# Autodesk Inventor assembly: Assembly_Cube_Z-Focus_Objective_v3
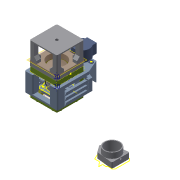
[picture p0: Inventor's stored thumbnail of the model, 180x180]
Saved by Autodesk Inventor 2019.4 (Build 234330000, 330)
## iProperties
Created: 2021-01-12
Part Number: Assembly_Cube_Z-Focus_Objective_v3
Document SubType Name: Assembly
Designer: diederichbenedict
Author: diederichbenedict
## Documents named in this file (5)
- C:\Users\diederichbenedict\Dropbox\Dokumente\Promotion\PROJECTS\UC2\02_CAD\INVENTOR\uc2_v3\Assembly_Cube_Z-Focus_Objective_v3.iam
- C:\Users\diederichbenedict\Dropbox\Dokumente\Promotion\PROJECTS\UC2\02_CAD\INVENTOR\uc2_v3\00_Olympus_40_1.3oil.ipt
- C:\Users\diederichbenedict\Dropbox\Dokumente\Promotion\PROJECTS\UC2\02_CAD\INVENTOR\uc2_v3\Assembly_Cube_Z_stage_sample_outercube_motorized.iam
- C:\Users\diederichbenedict\Dropbox\Dokumente\Promotion\PROJECTS\UC2\02_CAD\INVENTOR\uc2_v3\30_IM_SMAPLE_holder_v3.ipt
- C:\Users\diederichbenedict\Dropbox\Dokumente\Promotion\PROJECTS\UC2\02_CAD\INVENTOR\uc2_v3\30_IM_LED_holder_forcube_v3.ipt
## Components (4 placed, 4 different names)
1. 00_Olympus_40_1.3oil:1 — Insert:1
2. Assembly_Cube_Z_stage_sample_outercube_motorized:1 [sub-assembly] — Insert:1, Insert:2
3. 30_IM_SMAPLE_holder_v3:1 — Insert:2, Flush:1, Flush:2
4. 30_IM_LED_holder_forcube_v3:1 — Flush:1, Flush:2
## Relationships (4: Insert 2, Flush 2)
- Insert:1: 00_Olympus_40_1.3oil:1 ↔ Assembly_Cube_Z_stage_sample_outercube_motorized:1
- Insert:2: Assembly_Cube_Z_stage_sample_outercube_motorized:1 ↔ 30_IM_SMAPLE_holder_v3:1
- Flush:1: 30_IM_SMAPLE_holder_v3:1 ↔ 30_IM_LED_holder_forcube_v3:1
- Flush:2: 30_IM_SMAPLE_holder_v3:1 ↔ 30_IM_LED_holder_forcube_v3:1
